# Autodesk Inventor assembly: tube v
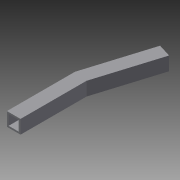
[picture p0: Inventor's stored thumbnail of the model, 180x180]
Saved by Autodesk Inventor 2013 (Build 170138000, 138)
## iProperties
Created: 2013-02-08
Part Number: tube v
Document SubType Name: Assembly
Designer: Arpan
Author: Arpan
## Documents named in this file (2)
- C:\Users\Moses\Documents\GitHub\frc2013CAD\Cimber actual\tube v.iam
- C:\Users\Moses\Documents\GitHub\frc2013CAD\Cimber actual\V tube.ipt
## Components (2 placed, 1 different names)
1. V tube:1 — Mate:1, Flush:1, Mate:2
2. V tube:2 — Mate:1, Flush:1, Mate:2
## Relationships (3: Mate 2, Flush 1)
- Mate:1: V tube:1 ↔ V tube:2
- Flush:1: V tube:1 ↔ V tube:2
- Mate:2: V tube:1 ↔ V tube:2
